# Autodesk Inventor assembly: Trash_Storage_Unit
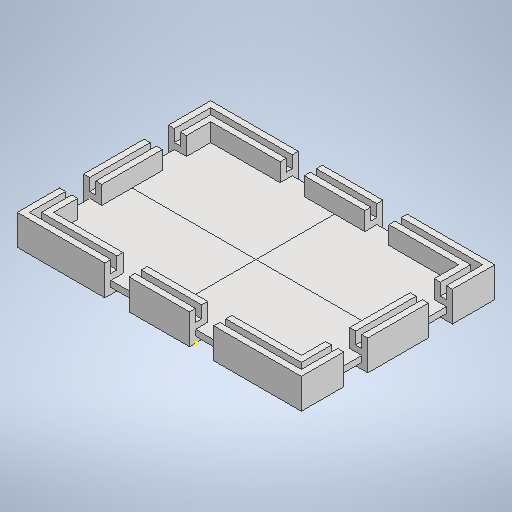
[picture p0: Inventor's stored thumbnail of the model, 512x512]
Saved by Autodesk Inventor 2025.2 (Build 292293000, 293)
## iProperties
Created: 2025-01-07
Part Number: Trash_Storage_Unit
Document SubType Name: Assembly
Designer: Matt Tidd
Author: Matt Tidd
## Documents named in this file (6)
- C:\Users\mtidd2\Desktop\H2A\CAD\TrashStorageUnit\Trash_Storage_Unit.iam
- C:\Users\mtidd2\Desktop\H2A\CAD\TrashStorageUnit\TSU_FM_Floor.ipt
- C:\Users\mtidd2\Desktop\H2A\CAD\TrashStorageUnit\TSU_MF_Floor.ipt
- C:\Users\mtidd2\Desktop\H2A\CAD\TrashStorageUnit\TSU_Y_Clamp.ipt
- C:\Users\mtidd2\Desktop\H2A\CAD\TrashStorageUnit\TSU_Corner1_Clamp.ipt
- C:\Users\mtidd2\Desktop\H2A\CAD\TrashStorageUnit\TSU_Corner2_Clamp.ipt
## Components (12 placed, 5 different names)
1. TSU_FM_Floor:1 — Mate:3, Mate:4, Mate:7, Mate:8, Mate:9, Mate:10, Mate:19, Mate:20
2. TSU_MF_Floor:1 — Mate:1, Mate:2, Mate:3, Mate:4, Mate:11, Mate:12, Mate:23, Mate:24
3. TSU_FM_Floor:2 — Mate:1, Mate:2, Mate:5, Mate:6, Mate:13, Mate:15, Mate:16
4. TSU_MF_Floor:2 — Mate:5, Mate:6, Mate:14, Mate:21, Mate:22
5. TSU_Y_Clamp:1 — Mate:7, Mate:8
6. TSU_Y_Clamp:2 — Mate:11, Mate:12
7. TSU_Y_Clamp:3 — Mate:13, Mate:14
8. TSU_Y_Clamp:4 — Mate:9, Mate:10
9. TSU_Corner1_Clamp:1 — Mate:21, Mate:22
10. TSU_Corner1_Clamp:2 — Mate:23, Mate:24
11. TSU_Corner2_Clamp:1 — Mate:15, Mate:16
12. TSU_Corner2_Clamp:2 — Mate:19, Mate:20
## Relationships (22: Mate 22)
- Mate:1: TSU_MF_Floor:1 ↔ TSU_FM_Floor:2
- Mate:2: TSU_MF_Floor:1 ↔ TSU_FM_Floor:2
- Mate:3: TSU_FM_Floor:1 ↔ TSU_MF_Floor:1
- Mate:4: TSU_FM_Floor:1 ↔ TSU_MF_Floor:1
- Mate:5: TSU_FM_Floor:2 ↔ TSU_MF_Floor:2
- Mate:6: TSU_FM_Floor:2 ↔ TSU_MF_Floor:2
- Mate:7: TSU_FM_Floor:1 ↔ TSU_Y_Clamp:1
- Mate:8: TSU_FM_Floor:1 ↔ TSU_Y_Clamp:1
- Mate:9: TSU_FM_Floor:1 ↔ TSU_Y_Clamp:4
- Mate:10: TSU_FM_Floor:1 ↔ TSU_Y_Clamp:4
- Mate:11: TSU_MF_Floor:1 ↔ TSU_Y_Clamp:2
- Mate:12: TSU_MF_Floor:1 ↔ TSU_Y_Clamp:2
- Mate:13: TSU_FM_Floor:2 ↔ TSU_Y_Clamp:3
- Mate:14: TSU_MF_Floor:2 ↔ TSU_Y_Clamp:3
- Mate:15: TSU_FM_Floor:2 ↔ TSU_Corner2_Clamp:1
- Mate:16: TSU_FM_Floor:2 ↔ TSU_Corner2_Clamp:1
- Mate:19: TSU_FM_Floor:1 ↔ TSU_Corner2_Clamp:2
- Mate:20: TSU_FM_Floor:1 ↔ TSU_Corner2_Clamp:2
- Mate:21: TSU_MF_Floor:2 ↔ TSU_Corner1_Clamp:1
- Mate:22: TSU_MF_Floor:2 ↔ TSU_Corner1_Clamp:1
- Mate:23: TSU_MF_Floor:1 ↔ TSU_Corner1_Clamp:2
- Mate:24: TSU_MF_Floor:1 ↔ TSU_Corner1_Clamp:2
